# Autodesk Inventor assembly: Wheel
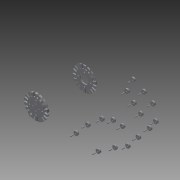
[picture p0: Inventor's stored thumbnail of the model, 180x180]
Saved by Autodesk Inventor 2015 (Build 190159000, 159)
## iProperties
Created: 2016-10-18
Part Number: Wheel
Document SubType Name: Assembly
Designer: James Yelland
Author: James Yelland
## Documents named in this file (7)
- C:\Users\James Yelland\git\LJ-STAND\Design\Models\Wheel\Wheel.iam
- C:\Users\James Yelland\git\LJ-STAND\Design\Models\Wheel\Plate 1.ipt
- C:\Users\James Yelland\git\LJ-STAND\Design\Models\Wheel\Plate 2.ipt
- C:\Users\James Yelland\git\LJ-STAND\Design\Models\Wheel\Plate 3.ipt
- C:\Users\James Yelland\git\LJ-STAND\Design\Models\Wheel\Rod.ipt
- C:\Users\James Yelland\git\LJ-STAND\Design\Models\Wheel\Wheel.ipt
- C:\Users\James Yelland\git\LJ-STAND\Design\Models\Wheel\Hub.ipt
## Components (40 placed, 6 different names)
1. Plate 1:1 — Insert:1, Insert:2, Tangent:1, Insert:3, Insert:4
2. Plate 2:1 — Insert:1, Insert:2, Mate:1, Tangent:2, Mate:3
3. Plate 3:1
4. Rod:1
5. Wheel:1
6. Rod:2
7. Wheel:2
8. Rod:3
9. Wheel:3
10. Rod:4
11. Wheel:4
12. Rod:5
13. Wheel:5
14. Rod:6
15. Wheel:6
16. Rod:7
17. Wheel:7
18. Rod:8
19. Wheel:8
20. Rod:9
21. Wheel:9
22. Rod:10
23. Wheel:10
24. Rod:11
25. Wheel:11
26. Rod:12
27. Wheel:12
28. Rod:13
29. Wheel:13
30. Rod:14
31. Wheel:14
32. Rod:15
33. Wheel:15
34. Rod:16
35. Wheel:16
36. Rod:17
37. Wheel:17
38. Rod:18 — Tangent:1, Mate:1, Tangent:2, Mate:2
39. Wheel:18 — Mate:2, Mate:3
40. Hub:1 — Insert:3, Insert:4
## Relationships (9: Insert 4, Mate 3, Tangent 2)
- Insert:1: Plate 1:1 ↔ Plate 2:1
- Insert:2: Plate 1:1 ↔ Plate 2:1
- Tangent:1: Plate 1:1 ↔ Rod:18
- Mate:1: Plate 2:1 ↔ Rod:18
- Tangent:2: Plate 2:1 ↔ Rod:18
- Mate:2: Rod:18 ↔ Wheel:18
- Mate:3 (0.1 mm): Plate 2:1 ↔ Wheel:18
- Insert:3: Plate 1:1 ↔ Hub:1
- Insert:4: Plate 1:1 ↔ Hub:1
